# Autodesk Inventor assembly: YAxisMotorRight
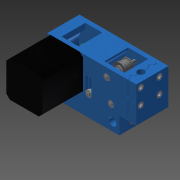
[picture p0: Inventor's stored thumbnail of the model, 180x180]
Saved by Autodesk Inventor 2015 (Build 190159000, 159)
## iProperties
Created: 2014-08-09
Part Number: YAxisMotorRight
Document SubType Name: Assembly
Designer: Jack
Author: Jack
## Documents named in this file (13)
- C:\Users\t_clevj\ownCloud\CoreXY\InventorModel\YAxis\YAxisMotorRight.iam
- C:\Users\t_clevj\ownCloud\CoreXY\InventorModel\YAxis\YAxisMotorBlockRight.ipt
- C:\Users\t_clevj\ownCloud\CoreXY\InventorModel\YAxis\YAxisMotorCapRight.ipt
- C:\Users\t_clevj\ownCloud\CoreXY\InventorModel\Hardware\Bolts\SHCS\SHCS5\SHCS5x10.ipt
- C:\Users\t_clevj\ownCloud\CoreXY\InventorModel\Hardware\Bolts\FHS\FHS5\5x10FHS.ipt
- C:\Users\t_clevj\ownCloud\CoreXY\InventorModel\Hardware\Bolts\SHCS\SHCS4\SHCS4x35.ipt
- C:\Users\t_clevj\ownCloud\CoreXY\InventorModel\Hardware\Bolts\SHCS\SHCS3\SHCS3x8.ipt
- C:\Users\t_clevj\ownCloud\CoreXY\InventorModel\Electronics\Motors\StepperMotorNema17.ipt
- C:\Users\t_clevj\ownCloud\CoreXY\InventorModel\Hardware\Bolts\SHCS\SHCS4\SHCS4x15.ipt
- C:\Users\t_clevj\ownCloud\CoreXY\InventorModel\Hardware\Nuts\Nut4.ipt
- C:\Users\t_clevj\ownCloud\CoreXY\InventorModel\Hardware\Belt\PulleyGT2x20tx5mmBore.ipt
- C:\Users\t_clevj\ownCloud\CoreXY\InventorModel\Hardware\Wahsers\M4Washer.ipt
- C:\Users\t_clevj\ownCloud\CoreXY\InventorModel\Hardware\Bearing\BearingRadialBall\BearingRadialBallF624zz.ipt
## Components (39 placed, 12 different names)
1. YAxisMotorBlockRight:1 — Mate:12, Flush:3, Mate:11, Flush:4, Flush:1, Mate:1, Mate:4, Mate:2, Mate:5, Mate:3, Mate:9, Mate:7, Mate:10, Mate:8, Flush:2, Mate:6, Mate:16, Mate:13, Mate:15, Mate:14, Mate:24, Mate:17, Mate:22, Mate:19, Mate:23, Mate:18, Mate:21, Mate:20, Mate:25, Angle:1, Mate:41, Angle:2, Mate:40, Angle:3, Mate:39, Slider:1, Mate:76, Mate:77, Mate:78, Flush:4, Angle:6, Angle:7, Angle:8, Angle:9, Mate:79, Mate:80, Mate:81, Mate:82
2. YAxisMotorCapRight:1 — Flush:4, Flush:1, Mate:1, Mate:34, Mate:30, Mate:35, Mate:31, Mate:33, Mate:29, Mate:32, Mate:28
3. StepperMotorNema17:1 — Mate:27, Mate:26, Mate:25, Mate:51
4. PulleyGT2x20tx5mmBore:1 — Mate:51, Flush:4
5. M4Washer:3
6. M4Washer:1
7. M4Washer:5
8. BearingRadialBallF624zz:6
9. BearingRadialBallF624zz:5
10. M4Washer:6 — Mate:75, Mate:77
11. BearingRadialBallF624zz:4
12. BearingRadialBallF624zz:3
13. M4Washer:4 — Mate:67, Mate:78
14. BearingRadialBallF624zz:2
15. BearingRadialBallF624zz:1
16. M4Washer:2 — Mate:59, Mate:76
17. Nut4:3 — Angle:1, Mate:41, Mate:36
18. Nut4:4 — Angle:2, Mate:40, Mate:37
19. Nut4:5 — Angle:3, Mate:39, Mate:38
20. SHCS4x35:2 — Mate:15, Mate:14, Mate:37, Mate:67
21. SHCS4x35:1 — Mate:16, Mate:13, Mate:36, Mate:59
22. SHCS4x35:3 — Mate:38, Slider:1, Mate:75
23. SHCS4x15:1 — Mate:34, Mate:30, Mate:44
24. SHCS4x15:2 — Mate:35, Mate:31, Mate:43
25. SHCS4x15:4 — Mate:32, Mate:28, Mate:46
26. SHCS4x15:3 — Mate:33, Mate:29, Mate:48
27. Nut4:7 — Mate:43, Angle:7, Mate:81
28. Nut4:6 — Mate:44, Angle:6, Mate:80
29. Nut4:2 — Mate:46, Angle:8, Mate:82
30. Nut4:1 — Mate:48, Angle:9, Mate:79
31. SHCS5x10:4 — Mate:10, Mate:8
32. SHCS5x10:3 — Mate:9, Mate:7
33. 5x10FHS:1 — Flush:2, Mate:6
34. SHCS5x10:1 — Mate:4, Mate:2
35. SHCS5x10:2 — Mate:5, Mate:3
36. SHCS3x8:1 — Mate:24, Mate:17, Mate:26
37. SHCS3x8:2 — Mate:22, Mate:19
38. SHCS3x8:3 — Mate:23, Mate:18, Mate:27
39. SHCS3x8:4 — Mate:21, Mate:20
## Relationships (87: Mate 75, Angle 7, Flush 4, TranslationJoint 1)
- Mate:12: YAxisMotorBlockRight:1
- Flush:3 [Mate]: YAxisMotorBlockRight:1
- Mate:11: YAxisMotorBlockRight:1
- Flush:4: YAxisMotorBlockRight:1 ↔ YAxisMotorCapRight:1
- Flush:1: YAxisMotorBlockRight:1 ↔ YAxisMotorCapRight:1
- Mate:1: YAxisMotorBlockRight:1 ↔ YAxisMotorCapRight:1
- Mate:4: YAxisMotorBlockRight:1 ↔ SHCS5x10:1
- Mate:2: YAxisMotorBlockRight:1 ↔ SHCS5x10:1
- Mate:5: YAxisMotorBlockRight:1 ↔ SHCS5x10:2
- Mate:3: YAxisMotorBlockRight:1 ↔ SHCS5x10:2
- Mate:9: YAxisMotorBlockRight:1 ↔ SHCS5x10:3
- Mate:7: YAxisMotorBlockRight:1 ↔ SHCS5x10:3
- Mate:10: YAxisMotorBlockRight:1 ↔ SHCS5x10:4
- Mate:8: YAxisMotorBlockRight:1 ↔ SHCS5x10:4
- Flush:2: YAxisMotorBlockRight:1 ↔ 5x10FHS:1
- Mate:6: YAxisMotorBlockRight:1 ↔ 5x10FHS:1
- Mate:16: YAxisMotorBlockRight:1 ↔ SHCS4x35:1
- Mate:13: YAxisMotorBlockRight:1 ↔ SHCS4x35:1
- Mate:15: YAxisMotorBlockRight:1 ↔ SHCS4x35:2
- Mate:14: YAxisMotorBlockRight:1 ↔ SHCS4x35:2
- Mate:24: YAxisMotorBlockRight:1 ↔ SHCS3x8:1
- Mate:17: YAxisMotorBlockRight:1 ↔ SHCS3x8:1
- Mate:22: YAxisMotorBlockRight:1 ↔ SHCS3x8:2
- Mate:19: YAxisMotorBlockRight:1 ↔ SHCS3x8:2
- Mate:23: YAxisMotorBlockRight:1 ↔ SHCS3x8:3
- Mate:18: YAxisMotorBlockRight:1 ↔ SHCS3x8:3
- Mate:21: YAxisMotorBlockRight:1 ↔ SHCS3x8:4
- Mate:20: YAxisMotorBlockRight:1 ↔ SHCS3x8:4
- Mate:27: StepperMotorNema17:1 ↔ SHCS3x8:3
- Mate:26: StepperMotorNema17:1 ↔ SHCS3x8:1
- Mate:25: YAxisMotorBlockRight:1 ↔ StepperMotorNema17:1
- Mate:34: YAxisMotorCapRight:1 ↔ SHCS4x15:1
- Mate:30: YAxisMotorCapRight:1 ↔ SHCS4x15:1
- Mate:35: YAxisMotorCapRight:1 ↔ SHCS4x15:2
- Mate:31: YAxisMotorCapRight:1 ↔ SHCS4x15:2
- Mate:33: YAxisMotorCapRight:1 ↔ SHCS4x15:3
- Mate:29: YAxisMotorCapRight:1 ↔ SHCS4x15:3
- Mate:32: YAxisMotorCapRight:1 ↔ SHCS4x15:4
- Mate:28: YAxisMotorCapRight:1 ↔ SHCS4x15:4
- Mate:48: SHCS4x15:3 ↔ Nut4:1
- Mate:46: SHCS4x15:4 ↔ Nut4:2
- Angle:1 (0 deg): YAxisMotorBlockRight:1 ↔ Nut4:3
- Mate:41: YAxisMotorBlockRight:1 ↔ Nut4:3
- Mate:36: Nut4:3 ↔ SHCS4x35:1
- Angle:2 (0 deg): YAxisMotorBlockRight:1 ↔ Nut4:4
- Mate:40: YAxisMotorBlockRight:1 ↔ Nut4:4
- Mate:37: Nut4:4 ↔ SHCS4x35:2
- Angle:3 (0 deg): YAxisMotorBlockRight:1 ↔ Nut4:5
- Mate:39: YAxisMotorBlockRight:1 ↔ Nut4:5
- Mate:38: Nut4:5 ↔ SHCS4x35:3
- Mate:44: SHCS4x15:1 ↔ Nut4:6
- Mate:43: SHCS4x15:2 ↔ Nut4:7
- Slider:1 [TranslationJoint]: YAxisMotorBlockRight:1 ↔ SHCS4x35:3
- Mate:51: StepperMotorNema17:1 ↔ PulleyGT2x20tx5mmBore:1
- [Mate]: BearingRadialBallF624zz:2 ↔ BearingRadialBallF624zz:1
- [Mate]: BearingRadialBallF624zz:2 ↔ BearingRadialBallF624zz:1
- [Mate]: M4Washer:1 ↔ BearingRadialBallF624zz:1
- [Mate]: M4Washer:1 ↔ BearingRadialBallF624zz:2
- [Mate]: BearingRadialBallF624zz:1 ↔ M4Washer:2
- [Mate]: BearingRadialBallF624zz:1 ↔ M4Washer:2
- Mate:59: M4Washer:2 ↔ SHCS4x35:1
- [Mate]: BearingRadialBallF624zz:4 ↔ BearingRadialBallF624zz:3
- [Mate]: BearingRadialBallF624zz:4 ↔ BearingRadialBallF624zz:3
- [Mate]: M4Washer:3 ↔ BearingRadialBallF624zz:3
- [Mate]: M4Washer:3 ↔ BearingRadialBallF624zz:4
- [Mate]: BearingRadialBallF624zz:3 ↔ M4Washer:4
- [Mate]: BearingRadialBallF624zz:3 ↔ M4Washer:4
- Mate:67: M4Washer:4 ↔ SHCS4x35:2
- [Mate]: BearingRadialBallF624zz:6 ↔ BearingRadialBallF624zz:5
- [Mate]: BearingRadialBallF624zz:6 ↔ BearingRadialBallF624zz:5
- [Mate]: M4Washer:5 ↔ BearingRadialBallF624zz:5
- [Mate]: M4Washer:5 ↔ BearingRadialBallF624zz:6
- [Mate]: BearingRadialBallF624zz:5 ↔ M4Washer:6
- [Mate]: BearingRadialBallF624zz:5 ↔ M4Washer:6
- Mate:75: M4Washer:6 ↔ SHCS4x35:3
- Mate:76 (9.4 mm): YAxisMotorBlockRight:1 ↔ M4Washer:2
- Mate:77 (9.4 mm): YAxisMotorBlockRight:1 ↔ M4Washer:6
- Mate:78 (9.4 mm): YAxisMotorBlockRight:1 ↔ M4Washer:4
- Flush:4 (-11.7 mm): YAxisMotorBlockRight:1 ↔ PulleyGT2x20tx5mmBore:1
- Angle:6 (0 deg): YAxisMotorBlockRight:1 ↔ Nut4:6
- Angle:7 (0 deg): YAxisMotorBlockRight:1 ↔ Nut4:7
- Angle:8 (0 deg): YAxisMotorBlockRight:1 ↔ Nut4:2
- Angle:9 (0 deg): YAxisMotorBlockRight:1 ↔ Nut4:1
- Mate:79: YAxisMotorBlockRight:1 ↔ Nut4:1
- Mate:80: YAxisMotorBlockRight:1 ↔ Nut4:6
- Mate:81: YAxisMotorBlockRight:1 ↔ Nut4:7
- Mate:82: YAxisMotorBlockRight:1 ↔ Nut4:2
## Named parameters: d105_d160 = 0 mm, d106_d161 = 0 mm, d107_d162 = 0 mm, d108_d163 = 0 mm, d109_d158 = 0 mm, d110_d159 = 0 mm, d113_d160 = 0 mm, d114_d161 = 0 mm, d115_d162 = 0 mm, d116_d163 = 0 mm, d117_d158 = 0 mm, d118_d159 = 0 mm
